# Autodesk Inventor assembly: dash
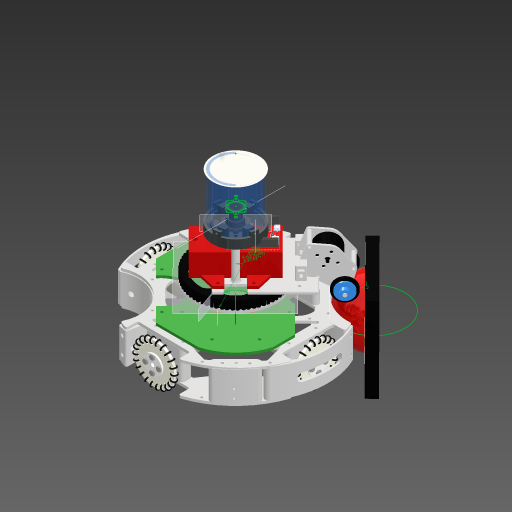
[picture p0: Inventor's stored thumbnail of the model, 512x512]
Saved by Autodesk Inventor 2023 (Build 270158000, 158)
## iProperties
Created: 2025-09-24
Part Number: dash
Document SubType Name: Assembly
Designer: daa
Author: daa
## Documents named in this file (6)
- C:\Users\daa\Documents\DASH_V2\omni_platforma\dash.iam
- C:\Users\daa\Documents\DASH_V2\omni_platforma\omni_platformav222.iam
- C:\Users\daa\Documents\DASH_V2\tower_V2.iam
- C:\Users\daa\Documents\DASH_V2\omni_platforma\plata_v2.ipt
- C:\Users\daa\Documents\DASH_V2\Dribler_v2\dribler_v2.iam
- C:\Users\daa\Documents\DASH_V2\ball_2.ipt
## Components (5 placed, 5 different names)
1. omni_platformav222:1 [sub-assembly] — Совмещение:1
2. plata_v2:1 — Совмещение:1, Совмещение:2
3. tower_V2:1 [sub-assembly] — Совмещение:2, С поворотом:1
4. ball_2:1
5. dribler_v2:1 [sub-assembly] — С поворотом:1
## Relationships (3: Mate 2, RevoluteJoint 1)
- Совмещение:1 [Mate]: omni_platformav222:1 ↔ plata_v2:1
- Совмещение:2 [Mate]: plata_v2:1 ↔ tower_V2:1
- С поворотом:1 [RevoluteJoint]: tower_V2:1 ↔ dribler_v2:1
